# Autodesk Inventor assembly: TubeHolderAssembly1
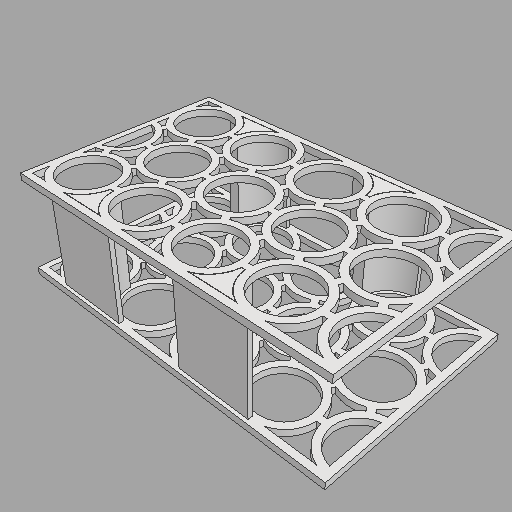
[picture p0: Inventor's stored thumbnail of the model, 512x512]
Saved by Autodesk Inventor 2025 (Build 290162010, 162A)
## iProperties
Created: 2025-03-07
Part Number: TubeHolderAssembly1
Document SubType Name: Assembly
Designer: schanen
Author: schanen
## Documents named in this file (2)
- H:\My Documents\3DPRINTS-GITHUB\3DPRINTS\TubeHolderAssembly1.iam
- H:\My Documents\3DPRINTS-GITHUB\3DPRINTS\TubeHolder.ipt
## Components (2 placed, 1 different names)
1. TubeHolder:1 — Flush:1, Flush:2, Flush:3
2. TubeHolder:2 — Flush:1, Flush:2, Flush:3
## Relationships (3: Flush 3)
- Flush:1: TubeHolder:1 ↔ TubeHolder:2
- Flush:2: TubeHolder:1 ↔ TubeHolder:2
- Flush:3: TubeHolder:1 ↔ TubeHolder:2
